# Autodesk Inventor assembly: Assembly_Matchboxscope_injectionmolded
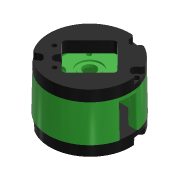
[picture p0: Inventor's stored thumbnail of the model, 180x180]
Saved by Autodesk Inventor 2022 (Build 260153000, 153)
## iProperties
Created: 2023-04-12
Part Number: Assembly_Matchboxscope_injectionmolded
Document SubType Name: Assembly
Designer: diederichbenedict
Author: diederichbenedict
## Documents named in this file (3)
- C:\Users\diederichbenedict\Dropbox\Dokumente\Promotion\PROJECTS\Matchboxscope\INVENTOR\RELEASE\Matchboxscope\Workspace\Assembly_Matchboxscope_injectionmolded.iam
- C:\Users\diederichbenedict\Dropbox\Dokumente\Promotion\PROJECTS\Matchboxscope\INVENTOR\RELEASE\Matchboxscope\Workspace\IM_Matchboxscope_base.ipt
- C:\Users\diederichbenedict\Dropbox\Dokumente\Promotion\PROJECTS\Matchboxscope\INVENTOR\RELEASE\Matchboxscope\Workspace\IM_Matchboxscope_plate.ipt
## Components (3 placed, 2 different names)
1. IM_Matchboxscope_base:1
2. IM_Matchboxscope_plate:1
3. IM_Matchboxscope_plate:2
## Relationships (4: Insert 3, Mate 1)
- [Insert]: IM_Matchboxscope_base:1 ↔ IM_Matchboxscope_plate:1
- [Insert]: IM_Matchboxscope_base:1 ↔ IM_Matchboxscope_plate:1
- [Insert]: IM_Matchboxscope_base:1 ↔ IM_Matchboxscope_plate:2
- [Mate]: IM_Matchboxscope_base:1 ↔ IM_Matchboxscope_plate:2
